# Autodesk Inventor assembly: SM-ZA02
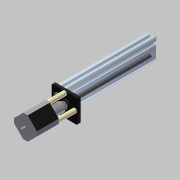
[picture p0: Inventor's stored thumbnail of the model, 180x180]
Saved by Autodesk Inventor 2012 SP1 (Build 160190100, 190)
## iProperties
Created: 2012-05-03
Part Number: SM-ZA02
Document SubType Name: Assembly
Designer: ERF
Stock Number: SM-ZA02
Author: ERF
Title: Z Axis Spindle Mount
## Documents named in this file (12)
- C:\Users\eford\Documents\Projects\Shapoko_v1i\Workspaces\Workspace\Projects\USER FOLDER\Edward\Shapeoko_v1i\Assemblies\SM-ZA02.iam
- C:\Users\eford\Documents\Projects\Shapoko_v1i\Workspaces\Workspace\Projects\USER FOLDER\Edward\Shapeoko_v1i\Parts\SM-S06.ipt
- C:\Users\eford\Documents\Projects\Shapoko_v1i\Workspaces\Workspace\Projects\USER FOLDER\Edward\Shapeoko_v1i\Parts\SM-H03.ipt
- C:\Users\eford\Documents\Projects\Shapoko_v1i\Workspaces\Workspace\Projects\USER FOLDER\Edward\Shapeoko_v1i\Parts\SM-H13.ipt
- C:\Users\eford\Documents\Projects\Shapoko_v1i\Workspaces\Workspace\Projects\USER FOLDER\Edward\Shapeoko_v1i\Parts\SM-M07.ipt
- C:\Users\eford\Documents\Projects\Shapoko_v1i\Workspaces\Workspace\Projects\USER FOLDER\Edward\Shapeoko_v1i\Parts\SM-H10.ipt
- C:\Users\eford\Documents\Projects\Shapoko_v1i\Workspaces\Workspace\Projects\USER FOLDER\Edward\Shapeoko_v1i\Parts\SM-H12.ipt
- C:\Users\eford\Documents\Projects\Shapoko_v1i\Workspaces\Workspace\Projects\USER FOLDER\Edward\Shapeoko_v1i\Parts\SM-H02.ipt
- C:\Users\eford\Documents\Projects\Shapoko_v1i\Workspaces\Workspace\Projects\USER FOLDER\Edward\Shapeoko_v1i\Parts\SM-E01.ipt
- C:\Users\eford\Documents\Projects\Shapoko_v1i\Workspaces\Workspace\Projects\USER FOLDER\Edward\Shapeoko_v1i\Parts\SM-H05.ipt
- C:\Users\eford\Documents\Projects\Shapoko_v1i\Workspaces\Workspace\Projects\USER FOLDER\Edward\Shapeoko_v1i\Parts\MSK01-03.ipt
- C:\Users\eford\Documents\Projects\Shapoko_v1i\Workspaces\Workspace\Projects\USER FOLDER\Edward\Shapeoko_v1i\Parts\SM-H06.ipt
## Components (21 placed, 11 different names)
1. SM-S06:1 — Mate:1, Flush:1, Insert:1, Insert:11, Insert:12, Insert:13, Insert:14, Insert:16, Insert:18, Angle:1
2. SM-H03:1 — Insert:5, Insert:6
3. SM-H13:1 — Insert:5
4. SM-M07:1 — Insert:1, Insert:3
5. SM-H10:1 — Insert:4, Insert:9
6. SM-H10:2 — Insert:3, Insert:4
7. SM-H12:1 — Insert:9
8. SM-H02:1 — Insert:14, Insert:15
9. SM-E01:1 — Insert:2, Mate:3, Insert:20, Angle:1
10. SM-H05:1 — Insert:2
11. MSK01-03:1 — Mate:1, Flush:1, Insert:6, Insert:8
12. SM-H13:2 — Insert:7
13. SM-H03:2 — Insert:7, Insert:8
14. SM-H06:1 — Insert:11, Mate:3
15. SM-H06:2 — Insert:12
16. SM-H06:3 — Insert:13
17. SM-H02:2 — Insert:15, Insert:20
18. SM-H02:3 — Insert:16, Insert:17
19. SM-H02:4 — Insert:17
20. SM-H02:5 — Insert:18, Insert:19
21. SM-H02:6 — Insert:19
## Relationships (23: Insert 19, Mate 2, Flush 1, Angle 1)
- Mate:1: SM-S06:1 ↔ MSK01-03:1
- Flush:1 (-5.4 mm): SM-S06:1 ↔ MSK01-03:1
- Insert:1: SM-S06:1 ↔ SM-M07:1
- Insert:2: SM-E01:1 ↔ SM-H05:1
- Insert:3: SM-M07:1 ↔ SM-H10:2
- Insert:4: SM-H10:1 ↔ SM-H10:2
- Insert:5: SM-H03:1 ↔ SM-H13:1
- Insert:6 (6.35 mm): SM-H03:1 ↔ MSK01-03:1
- Insert:7: SM-H13:2 ↔ SM-H03:2
- Insert:8 (6.35 mm): MSK01-03:1 ↔ SM-H03:2
- Insert:9: SM-H10:1 ↔ SM-H12:1
- Insert:11: SM-S06:1 ↔ SM-H06:1
- Insert:12: SM-S06:1 ↔ SM-H06:2
- Insert:13: SM-S06:1 ↔ SM-H06:3
- Mate:3: SM-E01:1 ↔ SM-H06:1
- Insert:14: SM-S06:1 ↔ SM-H02:1
- Insert:15: SM-H02:1 ↔ SM-H02:2
- Insert:16: SM-S06:1 ↔ SM-H02:3
- Insert:17: SM-H02:3 ↔ SM-H02:4
- Insert:18: SM-S06:1 ↔ SM-H02:5
- Insert:19: SM-H02:5 ↔ SM-H02:6
- Insert:20: SM-E01:1 ↔ SM-H02:2
- Angle:1 (0 deg): SM-S06:1 ↔ SM-E01:1
